# Autodesk Inventor assembly: Drivetrain Generator
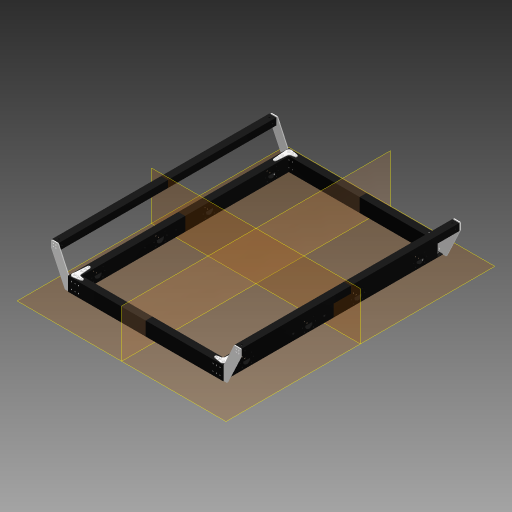
[picture p0: Inventor's stored thumbnail of the model, 512x512]
Saved by Autodesk Inventor 2023 (Build 270158000, 158)
## iProperties
RuleStatus: InUse
Created: 2022-02-12
Part Number: Drivetrain Generator
Document SubType Name: Assembly
Designer: Cal
Mass: 2624.05 g
Surface Area: 11929.1 cm^2
Volume: 971.872 cm^3
Density: 2.7 g/cm^3
Author: Cal
## Documents named in this file (6)
- E:\Collaborative Robots\Collaborative Part Library\Drivetrains\Generator\Drivetrain Generator.iam
- E:\Collaborative Robots\Collaborative Part Library\Drivetrains\Generator\Drivetrain Tubing.ipt
- E:\Collaborative Robots\Collaborative Part Library\Drivetrains\Generator\Drivetrain Tubing_MIR.ipt
- E:\Collaborative Robots\Collaborative Part Library\Drivetrains\VersaChassis Parts\VersaChassis Bumper Support Plate.ipt
- E:\Collaborative Robots\Collaborative Part Library\Hardware\Nuts and Threaded Blocks\WCP Tube Plug & Sleves.ipt
- E:\Collaborative Robots\Collaborative Part Library\Standard Custom Parts\Plates\Gussets\Gussets + Rivets.iam
## Components (18 placed, 5 different names)
1. Drivetrain Tubing:1 — Flush:1, Flush:2, Flush:3, Mate:1, Symmetry:1, Flush:5, Mate:2, Insert:16, Insert:17, Insert:20, Insert:21
2. Drivetrain Tubing_MIR:1 — Flush:1, Flush:2, Symmetry:1, Insert:14, Insert:15, Insert:18, Insert:19
3. Drivetrain Tubing:2 — Flush:3, Mate:1, Flush:4, Flush:5, Flush:6, Flush:7, Symmetry:2, Insert:3, Insert:4, Insert:7, Insert:8
4. Drivetrain Tubing:3 — Flush:6, Flush:7, Mate:2, Symmetry:2, Insert:1, Insert:2, Insert:5, Insert:6
5. VersaChassis Bumper Support Plate:1 — Insert:1, Insert:2, Flush:10, Insert:13
6. VersaChassis Bumper Support Plate:2 — Insert:3, Insert:4
7. VersaChassis Bumper Support Plate:3 — Insert:5, Insert:6
8. VersaChassis Bumper Support Plate:4 — Insert:7, Insert:8
9. Drivetrain Tubing:4 — Insert:9, Angle:1, Insert:10, Angle:2, Flush:8, Flush:9, Flush:10, Symmetry:3
10. WCP Tube Plug & Sleves:1 — Insert:9, Angle:1, Insert:13
11. WCP Tube Plug & Sleves:2 — Insert:10, Angle:2
12. Drivetrain Tubing:5 — Flush:8, Flush:9, Symmetry:3
13. WCP Tube Plug & Sleves:3
14. WCP Tube Plug & Sleves:4
15. Gussets + Rivets:1 [sub-assembly] — Insert:14, Insert:15
16. Gussets + Rivets:2 [sub-assembly] — Insert:16, Insert:17
17. Gussets + Rivets:3 [sub-assembly] — Insert:18, Insert:19
18. Gussets + Rivets:4 [sub-assembly] — Insert:20, Insert:21
## Relationships (40: Insert 21, Flush 10, Angle 4, Symmetry 3, Mate 2)
- Flush:1: Drivetrain Tubing:1 ↔ Drivetrain Tubing_MIR:1
- Flush:2: Drivetrain Tubing:1 ↔ Drivetrain Tubing_MIR:1
- Flush:3: Drivetrain Tubing:1 ↔ Drivetrain Tubing:2
- Mate:1: Drivetrain Tubing:1 ↔ Drivetrain Tubing:2
- Flush:4: Drivetrain Tubing:2
- Symmetry:1: Drivetrain Tubing:1 ↔ Drivetrain Tubing_MIR:1
- Flush:5: Drivetrain Tubing:1 ↔ Drivetrain Tubing:2
- Flush:6: Drivetrain Tubing:2 ↔ Drivetrain Tubing:3
- Flush:7: Drivetrain Tubing:2 ↔ Drivetrain Tubing:3
- Mate:2: Drivetrain Tubing:1 ↔ Drivetrain Tubing:3
- Symmetry:2: Drivetrain Tubing:2 ↔ Drivetrain Tubing:3
- Insert:1: Drivetrain Tubing:3 ↔ VersaChassis Bumper Support Plate:1
- Insert:2: Drivetrain Tubing:3 ↔ VersaChassis Bumper Support Plate:1
- Insert:3: Drivetrain Tubing:2 ↔ VersaChassis Bumper Support Plate:2
- Insert:4: Drivetrain Tubing:2 ↔ VersaChassis Bumper Support Plate:2
- Insert:5: Drivetrain Tubing:3 ↔ VersaChassis Bumper Support Plate:3
- Insert:6: Drivetrain Tubing:3 ↔ VersaChassis Bumper Support Plate:3
- Insert:7: Drivetrain Tubing:2 ↔ VersaChassis Bumper Support Plate:4
- Insert:8: Drivetrain Tubing:2 ↔ VersaChassis Bumper Support Plate:4
- Insert:9: Drivetrain Tubing:4 ↔ WCP Tube Plug & Sleves:1
- Angle:1 (0 deg): Drivetrain Tubing:4 ↔ WCP Tube Plug & Sleves:1
- Insert:10: Drivetrain Tubing:4 ↔ WCP Tube Plug & Sleves:2
- Angle:2 (0 deg): Drivetrain Tubing:4 ↔ WCP Tube Plug & Sleves:2
- [Insert]: Drivetrain Tubing:5 ↔ WCP Tube Plug & Sleves:3
- [Angle] (0 deg): Drivetrain Tubing:5 ↔ WCP Tube Plug & Sleves:3
- [Insert]: Drivetrain Tubing:5 ↔ WCP Tube Plug & Sleves:4
- [Angle] (0 deg): Drivetrain Tubing:5 ↔ WCP Tube Plug & Sleves:4
- Flush:8: Drivetrain Tubing:4 ↔ Drivetrain Tubing:5
- Flush:9: Drivetrain Tubing:4 ↔ Drivetrain Tubing:5
- Flush:10: VersaChassis Bumper Support Plate:1 ↔ Drivetrain Tubing:4
- Insert:13: VersaChassis Bumper Support Plate:1 ↔ WCP Tube Plug & Sleves:1
- Symmetry:3: Drivetrain Tubing:4 ↔ Drivetrain Tubing:5
- Insert:14: Drivetrain Tubing_MIR:1 ↔ Gussets + Rivets:1
- Insert:15: Drivetrain Tubing_MIR:1 ↔ Gussets + Rivets:1
- Insert:16: Drivetrain Tubing:1 ↔ Gussets + Rivets:2
- Insert:17: Drivetrain Tubing:1 ↔ Gussets + Rivets:2
- Insert:18: Drivetrain Tubing_MIR:1 ↔ Gussets + Rivets:3
- Insert:19: Drivetrain Tubing_MIR:1 ↔ Gussets + Rivets:3
- Insert:20: Drivetrain Tubing:1 ↔ Gussets + Rivets:4
- Insert:21: Drivetrain Tubing:1 ↔ Gussets + Rivets:4
## Named parameters: d21_d17 = 0 mm, d22_d18 = 0 deg, d23_d19 = 0 mm, d24_d20 = 0 deg
